# Autodesk Inventor assembly: Magnet_Assembly
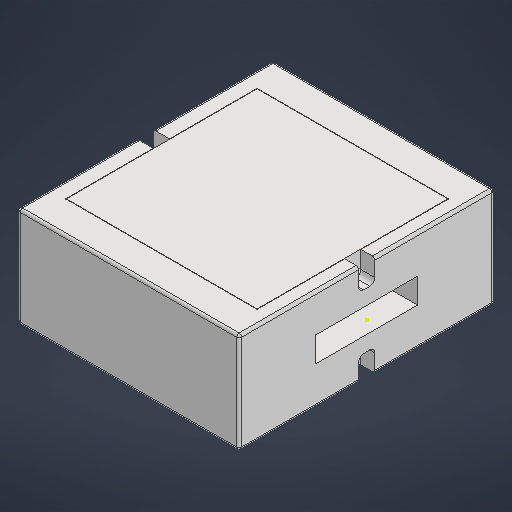
[picture p0: Inventor's stored thumbnail of the model, 512x512]
Saved by Autodesk Inventor 2026.2 (Build 302298000, 298)
## iProperties
Created: 2025-12-08
Part Number: Magnet_Assembly
Document SubType Name: Assembly
Designer: SCANTURK
Author: SCANTURK
## Documents named in this file (3)
- C:\Users\scanturk\OneDrive - University of South Carolina\Documents\GitHub\Compact-NMR\System_development\magnet_design\A320_Tesla_magnet\CAD\Magnet_Assembly.iam
- C:\Users\scanturk\OneDrive - University of South Carolina\Documents\GitHub\Compact-NMR\System_development\magnet_design\A320_Tesla_magnet\CAD\Base_Casing_A0320.ipt
- C:\Users\scanturk\OneDrive - University of South Carolina\Documents\GitHub\Compact-NMR\System_development\magnet_design\A320_Tesla_magnet\CAD\Sample_magnet_3_3_0.25.ipt
## Components (3 placed, 2 different names)
1. Base_Casing_A0320:1 — Mate:1, Mate:2, Flush:1, Mate:3, Mate:4, Flush:2
2. Sample_magnet_3_3_0.25:1 — Mate:1, Mate:2, Flush:1
3. Sample_magnet_3_3_0.25:2 — Mate:3, Mate:4, Flush:2
## Relationships (6: Mate 4, Flush 2)
- Mate:1 (0.15 mm): Base_Casing_A0320:1 ↔ Sample_magnet_3_3_0.25:1
- Mate:2 (0.15 mm): Base_Casing_A0320:1 ↔ Sample_magnet_3_3_0.25:1
- Flush:1: Base_Casing_A0320:1 ↔ Sample_magnet_3_3_0.25:1
- Mate:3 (0.15 mm): Base_Casing_A0320:1 ↔ Sample_magnet_3_3_0.25:2
- Mate:4: Base_Casing_A0320:1 ↔ Sample_magnet_3_3_0.25:2
- Flush:2: Base_Casing_A0320:1 ↔ Sample_magnet_3_3_0.25:2
